# Autodesk Inventor assembly: E002-Piston
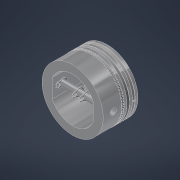
[picture p0: Inventor's stored thumbnail of the model, 180x180]
Saved by Autodesk Inventor 2021.3 (Build 253353000, 353)
## iProperties
Company: HES-SO
Created: 2022-03-31
Part Number: E002-Piston
Document SubType Name: Assembly
Designer: HER & ZAE
Mass: 20.147 g
Surface Area: 74.728 cm^2
Volume: 6.40419 cm^3
Density: 3.1459 g/cm^3
Author: HER & ZAE
## Documents named in this file (6)
- C:\Users\remi\OneDrive\Documents\Cours\05-HEVS\S2fb\mechanic\CCo\project\Compressor\E002-Piston.iam
- C:\Users\remi\OneDrive\Documents\Cours\05-HEVS\S2fb\mechanic\CCo\project\Compressor\P003-Corps_piston.ipt
- C:\Users\remi\OneDrive\Documents\Cours\05-HEVS\S2fb\mechanic\CCo\project\Compressor\P005-Axe_piston.ipt
- C:\Users\remi\OneDrive\Documents\Cours\05-HEVS\S2fb\mechanic\CCo\project\Compressor\Circlips\ungespannt_61799403.ipt
- C:\Users\remi\OneDrive\Documents\Cours\05-HEVS\S2fb\mechanic\CCo\project\Compressor\P027-Segment.ipt
- C:\Users\remi\OneDrive\Documents\Cours\05-HEVS\S2fb\mechanic\CCo\project\Compressor\P028-Segment_racleur.ipt
## Components (9 placed, 5 different names)
1. P003-Corps_piston:1 — Mate:1, Flush:1, Mate:10, Mate:11, Mate:12, Mate:13, Mate:14, Mate:15, Mate:16
2. P005-Axe_piston:1 — Mate:1, Flush:1, Mate:2, Mate:3, Mate:4, Mate:5, Mate:6, Mate:7, Mate:8, Mate:9
3. ungespannt_61799403:1 — Mate:2, Mate:4
4. ungespannt_61799403:2 — Mate:3, Mate:5
5. ungespannt_61799403:4 — Mate:6, Mate:9
6. ungespannt_61799403:5 — Mate:7, Mate:8
7. P027-Segment:1 — Mate:10, Mate:15, Mate:16, Angle:1
8. P027-Segment:2 — Mate:11, Mate:14, Angle:1, Angle:2
9. P028-Segment_racleur:1 — Mate:12, Mate:13, Angle:2
## Relationships (19: Mate 16, Angle 2, Flush 1)
- Mate:1: P003-Corps_piston:1 ↔ P005-Axe_piston:1
- Flush:1: P003-Corps_piston:1 ↔ P005-Axe_piston:1
- Mate:2: P005-Axe_piston:1 ↔ ungespannt_61799403:1
- Mate:3: P005-Axe_piston:1 ↔ ungespannt_61799403:2
- Mate:4: P005-Axe_piston:1 ↔ ungespannt_61799403:1
- Mate:5: P005-Axe_piston:1 ↔ ungespannt_61799403:2
- Mate:6: P005-Axe_piston:1 ↔ ungespannt_61799403:4
- Mate:7: P005-Axe_piston:1 ↔ ungespannt_61799403:5
- Mate:8: P005-Axe_piston:1 ↔ ungespannt_61799403:5
- Mate:9: P005-Axe_piston:1 ↔ ungespannt_61799403:4
- Mate:10: P003-Corps_piston:1 ↔ P027-Segment:1
- Mate:11: P003-Corps_piston:1 ↔ P027-Segment:2
- Mate:12: P003-Corps_piston:1 ↔ P028-Segment_racleur:1
- Mate:13: P003-Corps_piston:1 ↔ P028-Segment_racleur:1
- Mate:14: P003-Corps_piston:1 ↔ P027-Segment:2
- Mate:15: P003-Corps_piston:1 ↔ P027-Segment:1
- Mate:16: P003-Corps_piston:1 ↔ P027-Segment:1
- Angle:1 (120 deg): P027-Segment:1 ↔ P027-Segment:2
- Angle:2 (120 deg): P027-Segment:2 ↔ P028-Segment_racleur:1
